# Autodesk Inventor assembly: 书架装上滑台
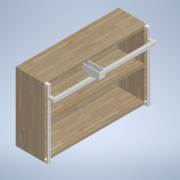
[picture p0: Inventor's stored thumbnail of the model, 180x180]
Saved by Autodesk Inventor 2020 (Build 240168000, 168)
## iProperties
Created: 2021-04-05
Part Number: 书架装上滑台
Document SubType Name: Assembly
Designer: 70929
Author: 70929
## Documents named in this file (6)
- D:\大创\图书整理机器人\建模\部件\书架装上滑台.iam
- D:\大创\图书整理机器人\建模\书架.ipt
- D:\大创\图书整理机器人\建模\竖直滑台.ipt
- D:\大创\图书整理机器人\建模\水平滑台.ipt
- D:\大创\图书整理机器人\建模\水平滑盖.ipt
- D:\大创\图书整理机器人\建模\滑盖上.ipt
## Components (6 placed, 5 different names)
1. 书架:1 — 配合:1, 配合:2, 配合:3, 配合:4, 配合:5, 配合:8
2. 竖直滑台:1 — 配合:1, 配合:2, 配合:3, 配合:6, 配合:7
3. 竖直滑台:2 — 配合:4, 配合:5, 配合:8
4. 水平滑台:1 — 配合:6, 配合:7, 配合:9, 配合:10
5. 水平滑盖:1 — 配合:9, 配合:10, 配合:11, 配合:12
6. 滑盖上:1 — 配合:11, 配合:12
## Relationships (12: Mate 12)
- 配合:1 [Mate]: 书架:1 ↔ 竖直滑台:1
- 配合:2 [Mate]: 书架:1 ↔ 竖直滑台:1
- 配合:3 [Mate]: 书架:1 ↔ 竖直滑台:1
- 配合:4 [Mate]: 书架:1 ↔ 竖直滑台:2
- 配合:5 [Mate]: 书架:1 ↔ 竖直滑台:2
- 配合:6 [Mate]: 竖直滑台:1 ↔ 水平滑台:1
- 配合:7 [Mate]: 竖直滑台:1 ↔ 水平滑台:1
- 配合:8 [Mate]: 书架:1 ↔ 竖直滑台:2
- 配合:9 [Mate]: 水平滑台:1 ↔ 水平滑盖:1
- 配合:10 [Mate]: 水平滑台:1 ↔ 水平滑盖:1
- 配合:11 [Mate]: 水平滑盖:1 ↔ 滑盖上:1
- 配合:12 [Mate]: 水平滑盖:1 ↔ 滑盖上:1
